# Autodesk Inventor assembly: Kiwi Robot
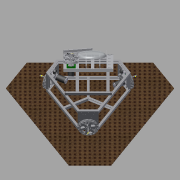
[picture p0: Inventor's stored thumbnail of the model, 180x180]
Saved by Autodesk Inventor 2013 (Build 170138000, 138)
## iProperties
Created: 2013-01-29
Part Number: Kiwi Robot
Document SubType Name: Assembly
Designer: carneeki
Author: carneeki
## Documents named in this file (7)
- C:\Autodesk\gruntmaster6000-cad\Kiwi Robot.iam
- C:\Autodesk\gruntmaster6000-cad\Chassis\Chassis.iam
- C:\Autodesk\gruntmaster6000-cad\Ground.ipt
- C:\Autodesk\gruntmaster6000-cad\Drive Wheel\Drive Wheel.iam
- C:\Autodesk\gruntmaster6000-cad\Rack\Rack.iam
- C:\Autodesk\gruntmaster6000-cad\Shooter\Shooter.iam
- C:\Autodesk\gruntmaster6000-cad\Shooter\Firing Mechanism.iam
## Components (8 placed, 6 different names)
1. Chassis:1 [sub-assembly] — Mate:1, Mate:2, Flush:1, Flush:2, Mate:3, Flush:3, Flush:4, Mate:4, Flush:5, Flush:6, Flush:9, Insert:1, Insert:2
2. Ground:1 — Mate:1, Flush:9
3. Rack:1 [sub-assembly] — Insert:1, Insert:2, Mate:6, Flush:11
4. Shooter:1 [sub-assembly] — Mate:6, Flush:11, Mate:7, Mate:8, Flush:12
5. Firing Mechanism:1 [sub-assembly] — Mate:7, Mate:8, Flush:12
6. Drive Wheel:1 [sub-assembly] — Mate:2, Flush:1, Flush:2
7. Drive Wheel:2 [sub-assembly] — Mate:4, Flush:5, Flush:6
8. Drive Wheel:3 [sub-assembly] — Mate:3, Flush:3, Flush:4
## Relationships (18: Flush 9, Mate 7, Insert 2)
- Mate:1 (38.1 mm): Chassis:1 ↔ Ground:1
- Mate:2: Chassis:1 ↔ Drive Wheel:1
- Flush:1: Chassis:1 ↔ Drive Wheel:1
- Flush:2: Chassis:1 ↔ Drive Wheel:1
- Mate:3: Chassis:1 ↔ Drive Wheel:3
- Flush:3: Chassis:1 ↔ Drive Wheel:3
- Flush:4: Chassis:1 ↔ Drive Wheel:3
- Mate:4: Chassis:1 ↔ Drive Wheel:2
- Flush:5: Chassis:1 ↔ Drive Wheel:2
- Flush:6: Chassis:1 ↔ Drive Wheel:2
- Flush:9 (254 mm): Chassis:1 ↔ Ground:1
- Insert:1: Chassis:1 ↔ Rack:1
- Insert:2: Chassis:1 ↔ Rack:1
- Mate:6: Rack:1 ↔ Shooter:1
- Flush:11: Rack:1 ↔ Shooter:1
- Mate:7 (25.4 mm): Shooter:1 ↔ Firing Mechanism:1
- Mate:8: Shooter:1 ↔ Firing Mechanism:1
- Flush:12: Shooter:1 ↔ Firing Mechanism:1
